# Autodesk Inventor assembly: Assembly2
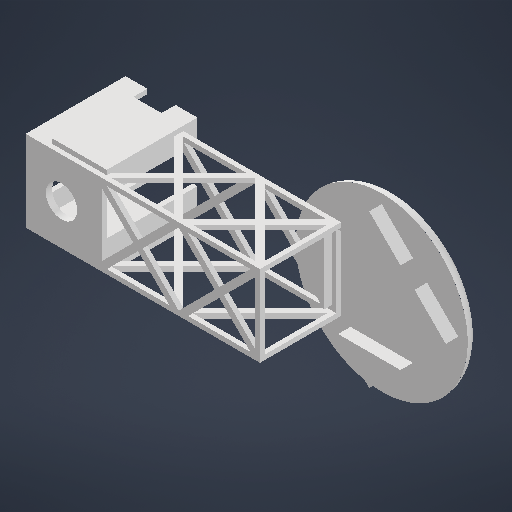
[picture p0: Inventor's stored thumbnail of the model, 512x512]
Saved by Autodesk Inventor 2026 (Build 300175000, 175)
## iProperties
Created: 2025-10-26
Part Number: Assembly2
Document SubType Name: Assembly
Designer: masak
Author: masak
## Documents named in this file (4)
- C:\Robohan\CAD\足回り\Assembly2.iam
- C:\Robohan\CAD\足回り\モーターホルダー試作.ipt
- C:\Robohan\CAD\足回り\足フレーム.ipt
- C:\Robohan\CAD\足回り\Part10.ipt
## Components (3 placed, 3 different names)
1. モーターホルダー試作:1 — フラッシュ:1
2. 足フレーム:1 — フラッシュ:1, フラッシュ:2
3. Part10:1 — フラッシュ:2
## Relationships (2: Flush 2)
- フラッシュ:1 [Flush]: モーターホルダー試作:1 ↔ 足フレーム:1
- フラッシュ:2 [Flush]: 足フレーム:1 ↔ Part10:1
